# Autodesk Inventor assembly: 810002_ASY-FAST ROVER v2
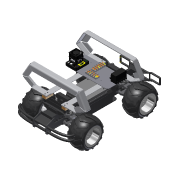
[picture p0: Inventor's stored thumbnail of the model, 180x180]
Saved by Autodesk Inventor 2015 (Build 190159000, 159)
## iProperties
Created: 2014-07-13
Part Number: 810002_ASY-FAST ROVER v2
Document SubType Name: Assembly
Designer: david
Author: david
## Documents named in this file (3)
- C:\SharedDrive\Dropbox\ICARUS\Rover\MECHANICAL\810002_ASY-FAST ROVER v2\810002_ASY-FAST ROVER v2.iam
- C:\SharedDrive\Dropbox\ICARUS\Rover\MECHANICAL\810002_ASY-FAST ROVER v2\813004_FAST ROVER v2 CHASSIS\813004_FAST ROVER v2 CHASSIS.iam
- C:\SharedDrive\Dropbox\ICARUS\Rover\MECHANICAL\810002_ASY-FAST ROVER v2\813006_FAST ROVER v2 CHASSIS ELECTRONICS\813006_FAST ROVER v2 CHASSIS ELECTRONICS.iam
## Components (2 placed, 2 different names)
1. 813004_FAST ROVER v2 CHASSIS:1 [sub-assembly] — Mate:1, Flush:1, Flush:2, Flush:3
2. 813006_FAST ROVER v2 CHASSIS ELECTRONICS:1 [sub-assembly] — Mate:1
## Relationships (4: Flush 3, Mate 1)
- Mate:1: 813004_FAST ROVER v2 CHASSIS:1 ↔ 813006_FAST ROVER v2 CHASSIS ELECTRONICS:1
- Flush:1: 813004_FAST ROVER v2 CHASSIS:1
- Flush:2: 813004_FAST ROVER v2 CHASSIS:1
- Flush:3: 813004_FAST ROVER v2 CHASSIS:1
